# Autodesk Inventor assembly: MeinbergTransmitter
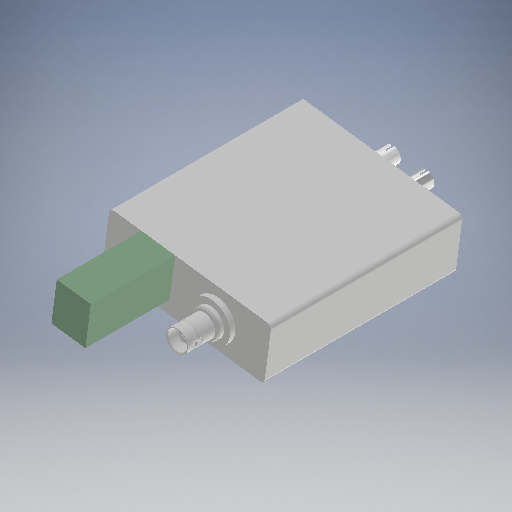
[picture p0: Inventor's stored thumbnail of the model, 512x512]
Saved by Autodesk Inventor 2025.3 (Build 293356000, 356)
## iProperties
Created: 2025-12-17
Part Number: MeinbergTransmitter
Document SubType Name: Assembly
Designer: sonata
Author: sonata
## Documents named in this file (5)
- D:\crush\RFoF\Parts\MeinbergTransmitter.iam
- D:\crush\RFoF-Meinberg\Parts\Meinberg_Box.ipt
- D:\crush\RFoF-Meinberg\Parts\a\a\a.ipt
- D:\crush\RFoF-Meinberg\Parts\ST Bulkhead ConnectorSLDPRT\ST Bulkhead ConnectorSLDPRT\ST Bulkhead ConnectorSLDPRT.ipt
- D:\crush\RFoF-Meinberg\Parts\MeinbergPower.ipt
## Components (5 placed, 4 different names)
1. Meinberg_Box:1 — Mate:1, Mate:2, Tangent:1, Tangent:2, Flush:1, Tangent:3, Mate:3, Tangent:4, Tangent:5, Mate:4, Flush:2, Flush:3
2. a:1 — Mate:1, Flush:1, Tangent:3
3. ST Bulkhead ConnectorSLDPRT:1 — Mate:2, Tangent:1, Tangent:2
4. ST Bulkhead ConnectorSLDPRT:2 — Mate:3, Tangent:4, Tangent:5
5. MeinbergPower:1 — Mate:4, Flush:2, Flush:3
## Relationships (12: Tangent 5, Mate 4, Flush 3)
- Mate:1: Meinberg_Box:1 ↔ a:1
- Mate:2: Meinberg_Box:1 ↔ ST Bulkhead ConnectorSLDPRT:1
- Tangent:1 (27 mm): Meinberg_Box:1 ↔ ST Bulkhead ConnectorSLDPRT:1
- Tangent:2 (11 mm): Meinberg_Box:1 ↔ ST Bulkhead ConnectorSLDPRT:1
- Flush:1 (15 mm): Meinberg_Box:1 ↔ a:1
- Tangent:3 (9 mm): Meinberg_Box:1 ↔ a:1
- Mate:3: Meinberg_Box:1 ↔ ST Bulkhead ConnectorSLDPRT:2
- Tangent:4 (11 mm): Meinberg_Box:1 ↔ ST Bulkhead ConnectorSLDPRT:2
- Tangent:5 (27 mm): Meinberg_Box:1 ↔ ST Bulkhead ConnectorSLDPRT:2
- Mate:4: Meinberg_Box:1 ↔ MeinbergPower:1
- Flush:2: Meinberg_Box:1 ↔ MeinbergPower:1
- Flush:3 (14 mm): Meinberg_Box:1 ↔ MeinbergPower:1
